# Autodesk Inventor assembly: Assemlby_TIRFImager_xyz_v0
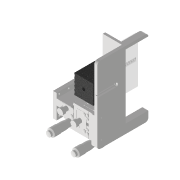
[picture p0: Inventor's stored thumbnail of the model, 180x180]
Saved by Autodesk Inventor 2022 (Build 260153000, 153)
## iProperties
Created: 2023-01-21
Part Number: Assemlby_TIRFImager_xyz_v0
Document SubType Name: Assembly
Designer: diederichbenedict
Author: diederichbenedict
## Documents named in this file (6)
- C:\Users\diederichbenedict\Dropbox\Dokumente\Promotion\PROJECTS\TIRFImager\INVENTOR\Assemlby_TIRFImager_xyz_v0.iam
- C:\Users\diederichbenedict\Dropbox\Dokumente\Promotion\PROJECTS\TIRFImager\INVENTOR\00_KES400.iam
- C:\Users\diederichbenedict\Dropbox\Dokumente\Promotion\PROJECTS\TIRFImager\INVENTOR\00_LASER_640nm.ipt
- C:\Users\diederichbenedict\Dropbox\Dokumente\Promotion\PROJECTS\TIRFImager\INVENTOR\00_XYZstage_micro_LT-4047-S1.ipt
- C:\Users\diederichbenedict\Dropbox\Dokumente\Promotion\PROJECTS\TIRFImager\INVENTOR\00_chipnano_waveguide_slidsize.ipt
- C:\Users\diederichbenedict\Dropbox\Dokumente\Promotion\PROJECTS\TIRFImager\INVENTOR\TIRFImager_base_xyz_v0.ipt
## Components (5 placed, 5 different names)
1. 00_KES400:1 [sub-assembly] — Einfügen:1, Passend:1, Passend:2
2. 00_LASER_640nm:1 — Einfügen:1, Fluchtend:2, Winkel:1, Fluchtend:3, Passend:3, Fluchtend:4, Fluchtend:7
3. 00_XYZstage_micro_LT-4047-S1:1 — Fluchtend:2, Fluchtend:3, Passend:3
4. 00_chipnano_waveguide_slidsize:1 — Passend:1, Winkel:1, Passend:2, Fluchtend:5, Fluchtend:6
5. TIRFImager_base_xyz_v0:1 — Winkel:2, Fluchtend:4, Fluchtend:5, Fluchtend:6, Fluchtend:7
## Relationships (13: Flush 7, Mate 3, Angle 2, Insert 1)
- [Flush]: 00_KES400:1 ↔ 00_LASER_640nm:1
- Einfügen:1 [Insert] (5 mm): 00_KES400:1 ↔ 00_LASER_640nm:1
- Fluchtend:2 [Flush] (5 mm): 00_LASER_640nm:1 ↔ 00_XYZstage_micro_LT-4047-S1:1
- Passend:1 [Mate]: 00_KES400:1 ↔ 00_chipnano_waveguide_slidsize:1
- Winkel:1 [Angle] (90 deg): 00_LASER_640nm:1 ↔ 00_chipnano_waveguide_slidsize:1
- Passend:2 [Mate] (3 mm): 00_KES400:1 ↔ 00_chipnano_waveguide_slidsize:1
- Fluchtend:3 [Flush] (-5 mm): 00_LASER_640nm:1 ↔ 00_XYZstage_micro_LT-4047-S1:1
- Passend:3 [Mate] (15 mm): 00_LASER_640nm:1 ↔ 00_XYZstage_micro_LT-4047-S1:1
- Winkel:2 [Angle] (0 deg): TIRFImager_base_xyz_v0:1
- Fluchtend:4 [Flush] (-5 mm): 00_LASER_640nm:1 ↔ TIRFImager_base_xyz_v0:1
- Fluchtend:5 [Flush] (10 mm): 00_chipnano_waveguide_slidsize:1 ↔ TIRFImager_base_xyz_v0:1
- Fluchtend:6 [Flush]: 00_chipnano_waveguide_slidsize:1 ↔ TIRFImager_base_xyz_v0:1
- Fluchtend:7 [Flush]: 00_LASER_640nm:1 ↔ TIRFImager_base_xyz_v0:1
